# Autodesk Inventor assembly: GANTRY
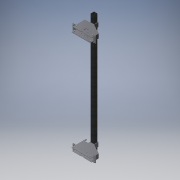
[picture p0: Inventor's stored thumbnail of the model, 180x180]
Saved by Autodesk Inventor 2018 (Build 220112000, 112)
## iProperties
Created: 2018-10-15
Part Number: GANTRY
Material: Genérico
Document SubType Name: Assembly
Designer: Toshiba
Author: Toshiba
## Documents named in this file (4)
- C:\U\Semestre Primavera 2018\Diseño de sistemas mecánicos\CNC\DiseñoCNC\Gantry\GANTRY.iam
- C:\U\Semestre Primavera 2018\Diseño de sistemas mecánicos\CNC\DiseñoCNC\Gantry\2350 STEEL PROFILE.ipt
- C:\U\Semestre Primavera 2018\Diseño de sistemas mecánicos\CNC\DiseñoCNC\Gantry\RIGHT RAIL ASSY.iam
- C:\U\Semestre Primavera 2018\Diseño de sistemas mecánicos\CNC\DiseñoCNC\Gantry\LEFT RAIL ASSY.iam
## Components (3 placed, 3 different names)
1. 2350 STEEL PROFILE:1 — Coincidencia:1, Coincidencia:2, Coincidencia:3, Coincidencia:4, Coincidencia:5, Coincidencia:6
2. RIGHT RAIL ASSY:1 [sub-assembly] — Coincidencia:1, Coincidencia:2, Coincidencia:5
3. LEFT RAIL ASSY:1 [sub-assembly] — Coincidencia:3, Coincidencia:4, Coincidencia:6
## Relationships (6: Mate 6)
- Coincidencia:1 [Mate]: 2350 STEEL PROFILE:1 ↔ RIGHT RAIL ASSY:1
- Coincidencia:2 [Mate]: 2350 STEEL PROFILE:1 ↔ RIGHT RAIL ASSY:1
- Coincidencia:3 [Mate]: 2350 STEEL PROFILE:1 ↔ LEFT RAIL ASSY:1
- Coincidencia:4 [Mate]: 2350 STEEL PROFILE:1 ↔ LEFT RAIL ASSY:1
- Coincidencia:5 [Mate] (154 mm): 2350 STEEL PROFILE:1 ↔ RIGHT RAIL ASSY:1
- Coincidencia:6 [Mate] (154 mm): 2350 STEEL PROFILE:1 ↔ LEFT RAIL ASSY:1
